# Autodesk Inventor assembly: extension arm spool 2_75 with sprocket
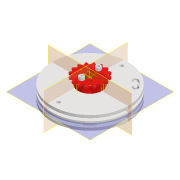
[picture p0: Inventor's stored thumbnail of the model, 180x180]
Saved by Autodesk Inventor 2020 (Build 240168000, 168)
## iProperties
Created: 2020-01-31
Part Number: extension arm spool 2_75 with sprocket
Document SubType Name: Assembly
Designer: ball
Author: ball
## Documents named in this file (7)
- C:\FTC\FTC8863CAD\2019 Robot\Delivery\extension arm\extension arm spool 2_75 with sprocket.iam
- C:\FTC\FTC8863CAD\2019 Robot\Delivery\extension arm\extension arm spool 2_75.iam
- C:\FTC\FTC8863CAD\2019 Robot\Delivery\extension arm\16 tooth sprocket mount on custom clamping hub.iam
- C:\FTC\FTC8863CAD\StepLibraries\Nuts\6-32 NYLON-INSERT LOCKNUT.ipt
- C:\FTC\FTC8863CAD\StepLibraries\Screws\6-32 x 1.250 SOCKET HEAD CAP SCREW.ipt
- C:\FTC\FTC8863CAD\Actobotics\633 parts\633104.ipt
- C:\FTC\FTC8863CAD\Actobotics\535 parts\535042.ipt
## Components (9 placed, 6 different names)
1. extension arm spool 2_75:1 [sub-assembly] — Mate:1, Mate:2, Mate:3, Mate:4, Mate:5, Mate:6, Mate:7, Mate:12, Mate:13, Mate:15, Flush:1
2. 16 tooth sprocket mount on custom clamping hub:1 [sub-assembly] — Mate:1, Mate:2, Mate:3, Mate:8, Mate:9, Mate:10, Mate:11
3. 6-32 NYLON-INSERT LOCKNUT:2 — Mate:4, Mate:5
4. 6-32 NYLON-INSERT LOCKNUT:3 — Mate:6, Mate:7
5. 6-32 x 1.250 SOCKET HEAD CAP SCREW:1 — Mate:8, Mate:10
6. 6-32 x 1.250 SOCKET HEAD CAP SCREW:2 — Mate:9, Mate:11
7. 633104:1 — Mate:12, Mate:13, Mate:16, Mate:17
8. 535042:1 — Mate:15, Mate:18, Mate:19
9. 633104:2 — Mate:16, Mate:17, Mate:18, Mate:19
## Relationships (19: Mate 18, Flush 1)
- Mate:1: extension arm spool 2_75:1 ↔ 16 tooth sprocket mount on custom clamping hub:1
- Mate:2: extension arm spool 2_75:1 ↔ 16 tooth sprocket mount on custom clamping hub:1
- Mate:3: extension arm spool 2_75:1 ↔ 16 tooth sprocket mount on custom clamping hub:1
- Mate:4: extension arm spool 2_75:1 ↔ 6-32 NYLON-INSERT LOCKNUT:2
- Mate:5: extension arm spool 2_75:1 ↔ 6-32 NYLON-INSERT LOCKNUT:2
- Mate:6: extension arm spool 2_75:1 ↔ 6-32 NYLON-INSERT LOCKNUT:3
- Mate:7: extension arm spool 2_75:1 ↔ 6-32 NYLON-INSERT LOCKNUT:3
- Mate:8: 16 tooth sprocket mount on custom clamping hub:1 ↔ 6-32 x 1.250 SOCKET HEAD CAP SCREW:1
- Mate:9: 16 tooth sprocket mount on custom clamping hub:1 ↔ 6-32 x 1.250 SOCKET HEAD CAP SCREW:2
- Mate:10: 16 tooth sprocket mount on custom clamping hub:1 ↔ 6-32 x 1.250 SOCKET HEAD CAP SCREW:1
- Mate:11: 16 tooth sprocket mount on custom clamping hub:1 ↔ 6-32 x 1.250 SOCKET HEAD CAP SCREW:2
- Mate:12: extension arm spool 2_75:1 ↔ 633104:1
- Mate:13: extension arm spool 2_75:1 ↔ 633104:1
- Mate:15: extension arm spool 2_75:1 ↔ 535042:1
- Mate:16: 633104:1 ↔ 633104:2
- Mate:17: 633104:1 ↔ 633104:2
- Mate:18: 535042:1 ↔ 633104:2
- Mate:19: 535042:1 ↔ 633104:2
- Flush:1 (-7.9375 mm): extension arm spool 2_75:1
